# Autodesk Inventor assembly: FULL ARM
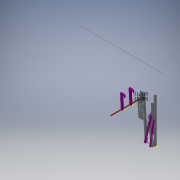
[picture p0: Inventor's stored thumbnail of the model, 180x180]
Saved by Autodesk Inventor 2016 (Build 200138000, 138)
## iProperties
Created: 2016-02-17
Part Number: FULL ARM
Document SubType Name: Weldment
Designer: Admin
Weld Material: Welded Aluminum-6061
Author: Admin
## Documents named in this file (18)
- C:\Users\matth_000\Desktop\Extra Pieces\FULL ARM.iam
- C:\Users\matth_000\Desktop\Arm_Lifter-2016-03-19\Arm Lifter\AP 1.ipt
- C:\Users\matth_000\Desktop\Arm_Lifter-2016-03-19\Arm Lifter\AP 2.ipt
- C:\Users\matth_000\Desktop\Arm_Lifter-2016-03-19\Arm Lifter\AP 3.ipt
- C:\Users\matth_000\Desktop\Arm_Lifter-2016-03-19\Arm Lifter\AP 4.ipt
- C:\Users\matth_000\Desktop\Arm_Lifter-2016-03-19\Arm Lifter\AP 5.ipt
- C:\Users\matth_000\Desktop\Arm_Lifter-2016-03-19\Arm Lifter\AP 6.ipt
- C:\Users\matth_000\Desktop\Arm_Lifter-2016-03-19\Arm Lifter\Plate.ipt
- C:\Users\matth_000\Desktop\Arm_Lifter-2016-03-19\Arm Lifter\Plate add on.ipt
- C:\Users\matth_000\Desktop\Arm_Lifter-2016-03-19\Arm Lifter\Hex Shaft.ipt
- C:\Users\matth_000\Desktop\Arm_Lifter-2016-03-19\Arm Lifter\claw.ipt
- C:\Users\matth_000\Desktop\Arm_Lifter-2016-03-19\Arm Lifter\motor and screw.ipt
- C:\Users\matth_000\Desktop\Arm_Lifter-2016-03-19\Arm Lifter\motor spinner.ipt
- C:\Users\matth_000\Desktop\Arm_Lifter-2016-03-19\Arm Lifter\Spinner.ipt
- C:\Users\matth_000\Desktop\Arm Lifter\AP 9.ipt
- C:\Users\matth_000\Desktop\Arm Lifter\AP 10.ipt
- C:\Users\matth_000\Desktop\Arm Lifter\meh.ipt
- C:\Users\matth_000\Desktop\Extra Pieces\meh2.ipt
## Components (18 placed, 17 different names)
1. AP 1:1 — Flush:1, Flush:2, Mate:2, Mate:19, Flush:3, Mate:34, Mate:41, Mate:56, Mate:64, Mate:69, Mate:72, Mate:76, Flush:12, Flush:13
2. AP 2:1 — Flush:3, Mate:32, Mate:73, Mate:79
3. AP 3:1 — Flush:2, Mate:36, Flush:4, Flush:5, Mate:71, Mate:81
4. AP 4:1 — Flush:1, Mate:35, Mate:78, Mate:80
5. AP 5:1 — Mate:2, Mate:19, Mate:32, Mate:78
6. AP 6:1 — Mate:34, Mate:35, Mate:41
7. Plate:1 — Mate:36, Flush:4, Flush:5, Flush:8, Mate:37, Flush:9
8. Plate add on:1 — Flush:8, Mate:37, Flush:9, Mate:38, Mate:39, Flush:10, Mate:46, Mate:77
9. Hex Shaft:1 — Mate:38, Mate:39, Flush:10, Mate:57, Mate:60, Mate:61, Mate:67, Mate:77
10. claw:1 — Mate:49, Mate:60, Mate:61
11. claw:2 — Mate:46, Mate:49, Mate:57, Mate:67
12. motor and screw:1 — Mate:65, Flush:11
13. motor spinner:1 — Mate:63, Mate:64, Mate:65, Flush:11, Mate:66
14. Spinner:1 — Mate:56, Mate:63, Mate:66
15. AP 9:1 — Mate:69, Mate:71, Mate:79
16. AP 10:1 — Mate:72, Mate:73, Mate:80, Mate:81
17. meh:1 — Mate:76, Flush:12, Flush:13
18. meh2:1
## Relationships (42: Mate 31, Flush 11)
- Flush:1: AP 1:1 ↔ AP 4:1
- Flush:2: AP 1:1 ↔ AP 3:1
- Mate:2 (6.35 mm): AP 1:1 ↔ AP 5:1
- Mate:19: AP 1:1 ↔ AP 5:1
- Flush:3: AP 1:1 ↔ AP 2:1
- Mate:32: AP 2:1 ↔ AP 5:1
- Mate:34: AP 1:1 ↔ AP 6:1
- Mate:35: AP 4:1 ↔ AP 6:1
- Mate:36: AP 3:1 ↔ Plate:1
- Flush:4: AP 3:1 ↔ Plate:1
- Flush:5: AP 3:1 ↔ Plate:1
- Flush:8: Plate:1 ↔ Plate add on:1
- Mate:37: Plate:1 ↔ Plate add on:1
- Flush:9: Plate:1 ↔ Plate add on:1
- Mate:38: Plate add on:1 ↔ Hex Shaft:1
- Mate:39: Plate add on:1 ↔ Hex Shaft:1
- Flush:10 (-25.4 mm): Plate add on:1 ↔ Hex Shaft:1
- Mate:41: AP 1:1 ↔ AP 6:1
- Mate:46 (127 mm): Plate add on:1 ↔ claw:2
- Mate:49 (118.618 mm): claw:1 ↔ claw:2
- Mate:56: AP 1:1 ↔ Spinner:1
- Mate:57: Hex Shaft:1 ↔ claw:2
- Mate:60: Hex Shaft:1 ↔ claw:1
- Mate:61: Hex Shaft:1 ↔ claw:1
- Mate:63: motor spinner:1 ↔ Spinner:1
- Mate:64: AP 1:1 ↔ motor spinner:1
- Mate:65: motor and screw:1 ↔ motor spinner:1
- Flush:11 (-25.4 mm): motor and screw:1 ↔ motor spinner:1
- Mate:66: motor spinner:1 ↔ Spinner:1
- Mate:67: Hex Shaft:1 ↔ claw:2
- Mate:69 (6.35 mm): AP 1:1 ↔ AP 9:1
- Mate:71: AP 3:1 ↔ AP 9:1
- Mate:72 (6.35 mm): AP 1:1 ↔ AP 10:1
- Mate:73: AP 2:1 ↔ AP 10:1
- Mate:76 (381 mm): AP 1:1 ↔ meh:1
- Flush:12: AP 1:1 ↔ meh:1
- Flush:13 (-101.6 mm): AP 1:1 ↔ meh:1
- Mate:77: Plate add on:1 ↔ Hex Shaft:1
- Mate:78: AP 4:1 ↔ AP 5:1
- Mate:79: AP 2:1 ↔ AP 9:1
- Mate:80: AP 4:1 ↔ AP 10:1
- Mate:81: AP 3:1 ↔ AP 10:1
